# Autodesk Inventor assembly: v2
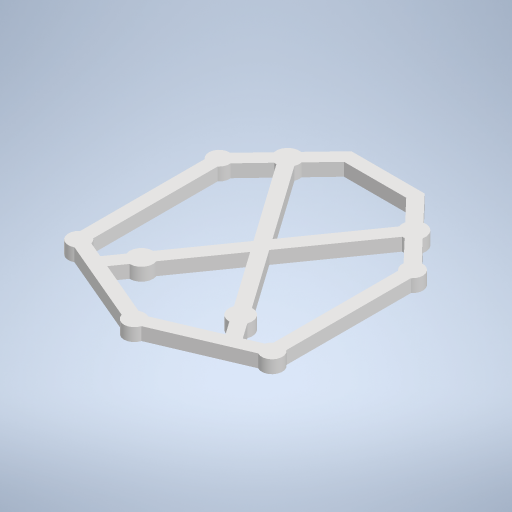
[picture p0: Inventor's stored thumbnail of the model, 512x512]
Saved by Autodesk Inventor 2024.2 (Build 282272000, 272)
## iProperties
Created: 2024-01-18
Part Number: v2
Document SubType Name: Assembly
Designer: Eric
Author: Eric
## Documents named in this file (3)
- C:\Users\Eric\Desktop\scioly-robot-tour\Hardware\ipt\v3\v3.iam
- C:\Users\Eric\Desktop\scioly-robot-tour\Hardware\ipt\v3\v3chassis.ipt
- C:\Users\Eric\Desktop\scioly-robot-tour\Hardware\ipt\v3\v3topframe.ipt
## Components (2 placed, 2 different names)
1. v3chassis:1 — Flush:1
2. v3topframe:1 — Flush:1
## Relationships (1: Flush 1)
- Flush:1 (19 mm): v3chassis:1 ↔ v3topframe:1
